# Autodesk Inventor assembly: F_Foot
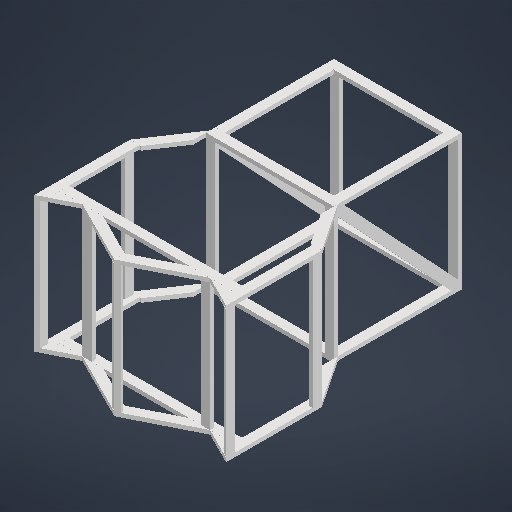
[picture p0: Inventor's stored thumbnail of the model, 512x512]
Saved by Autodesk Inventor 2027.1 (Build 311270010, 270A)
## iProperties
Created: 2025-09-08
Part Number: F_Foot
Document SubType Name: Assembly
Designer: trott
Author: trott
## Documents named in this file (11)
- C:\Users\jorda\OneDrive\Documents\GitHub\USC-ASME-TigerBurn-2026\CAD\Legs\Front Foot\F_Foot.iam
- C:\Users\jorda\OneDrive\Documents\GitHub\USC-ASME-TigerBurn-2026\CAD\Legs\Front Foot\2x4x48.ipt
- C:\Users\jorda\OneDrive\Documents\GitHub\USC-ASME-TigerBurn-2026\CAD\Legs\Front Foot\2x4x41.ipt
- C:\Users\jorda\OneDrive\Documents\GitHub\USC-ASME-TigerBurn-2026\CAD\Legs\Front Foot\2x4x65.ipt
- C:\Users\jorda\OneDrive\Documents\GitHub\USC-ASME-TigerBurn-2026\CAD\Legs\Front Foot\S_2x4x36.ipt
- C:\Users\jorda\OneDrive\Documents\GitHub\USC-ASME-TigerBurn-2026\CAD\Legs\Front Foot\S_2x4x9.503.ipt
- C:\Users\jorda\OneDrive\Documents\GitHub\USC-ASME-TigerBurn-2026\CAD\Legs\Front Foot\S_2x4x26.833.ipt
- C:\Users\jorda\OneDrive\Documents\GitHub\USC-ASME-TigerBurn-2026\CAD\Legs\Front Foot\S2_2x4x48.ipt
- C:\Users\jorda\OneDrive\Documents\GitHub\USC-ASME-TigerBurn-2026\CAD\Legs\Front Foot\S_2x4x48.ipt
- C:\Users\jorda\OneDrive\Documents\GitHub\USC-ASME-TigerBurn-2026\CAD\Legs\Front Foot\S_2x4x21.633.ipt
- C:\Users\jorda\OneDrive\Documents\GitHub\USC-ASME-TigerBurn-2026\CAD\Legs\Front Foot\S_2x4x65.795.ipt
## Components (39 placed, 10 different names)
1. 2x4x48:7 — Mate:17, Flush:23, Flush:24
2. 2x4x48:8 — Mate:18, Flush:25, Flush:26
3. S2_2x4x48:1 — Mate:19, Flush:27, Flush:28
4. S_2x4x48:1
5. S_2x4x48:2
6. 2x4x48:9 — Mate:39
7. 2x4x48:10 — Mate:36, Flush:54, Mate:42, Flush:55, Flush:56, Flush:57, Mate:43
8. S_2x4x65.795:1 — Mate:36
9. S_2x4x65.795:2 — Mate:39
10. 2x4x48:11 — Flush:54, Mate:42, Flush:55, Mate:46, Flush:62, Flush:63, Mate:47, Flush:64, Flush:65
11. 2x4x48:12 — Flush:56, Flush:57, Mate:43
12. 2x4x48:13 — Mate:44, Flush:58, Flush:59
13. 2x4x48:14 — Mate:45, Flush:60, Flush:61
14. 2x4x48:2 — Mate:44, Flush:58, Flush:59, Mate:45, Flush:60
15. 2x4x48:3
16. 2x4x48:4 — Mate:20, Flush:61
17. 2x4x48:5 — Mate:22
18. S_2x4x21.633:1
19. S_2x4x21.633:2
20. S_2x4x21.633:3
21. S_2x4x21.633:4 — Mate:20, Flush:29
22. 2x4x41:2 — Mate:47, Flush:64, Flush:65
23. 2x4x41:1 — Mate:46, Flush:62, Flush:63
24. S_2x4x36:2 — Mate:10, Flush:18, Mate:18, Flush:25, Flush:26, Flush:29, Mate:40, Flush:53
25. 2x4x65:1 — Mate:40, Flush:53, Mate:41
26. S_2x4x9.503:2 — Mate:10, Flush:18, Mate:22, Mate:41
27. S_2x4x26.833:2 — Mate:14, Flush:27
28. S_2x4x26.833:1 — Mate:13, Mate:14, Mate:19, Flush:28
29. S_2x4x9.503:1 — Mate:8, Flush:17, Mate:13
30. S_2x4x36:1 — Mate:8, Flush:17, Mate:17, Flush:23, Flush:24
31. 2x4x41:3
32. 2x4x41:4
33. S_2x4x36:3
34. 2x4x65:2
35. S_2x4x9.503:3
36. S_2x4x26.833:3
37. S_2x4x26.833:4
38. S_2x4x9.503:4
39. S_2x4x36:4
## Component patterns: (4 elements, first: 2x4x48:2), (2 elements, first: S_2x4x21.633:1 + S_2x4x21.633:2), (2 elements, first: 2x4x41:2 + 2x4x41:1 + S_2x4x36:2 + 2x4x65:1 + S_2x4x9.503:2 + S_2x4x26.833:2 + S_2x4x26.833:1 + S_2x4x9.503:1 + S_2x4x36:1)
## Relationships (41: Flush 22, Mate 19)
- Mate:8: S_2x4x9.503:1 ↔ S_2x4x36:1
- Flush:17: S_2x4x9.503:1 ↔ S_2x4x36:1
- Mate:10: S_2x4x36:2 ↔ S_2x4x9.503:2
- Flush:18: S_2x4x36:2 ↔ S_2x4x9.503:2
- Mate:13: S_2x4x26.833:1 ↔ S_2x4x9.503:1
- Mate:14: S_2x4x26.833:2 ↔ S_2x4x26.833:1
- Mate:17: 2x4x48:7 ↔ S_2x4x36:1
- Flush:23: 2x4x48:7 ↔ S_2x4x36:1
- Flush:24: 2x4x48:7 ↔ S_2x4x36:1
- Mate:18: 2x4x48:8 ↔ S_2x4x36:2
- Flush:25: 2x4x48:8 ↔ S_2x4x36:2
- Flush:26: 2x4x48:8 ↔ S_2x4x36:2
- Mate:19: S2_2x4x48:1 ↔ S_2x4x26.833:1
- Flush:27: S2_2x4x48:1 ↔ S_2x4x26.833:2
- Flush:28: S2_2x4x48:1 ↔ S_2x4x26.833:1
- Mate:20: 2x4x48:4 ↔ S_2x4x21.633:4
- Flush:29: S_2x4x21.633:4 ↔ S_2x4x36:2
- Mate:22: 2x4x48:5 ↔ S_2x4x9.503:2
- Mate:36: 2x4x48:10 ↔ S_2x4x65.795:1
- Mate:39: 2x4x48:9 ↔ S_2x4x65.795:2
- Mate:40: S_2x4x36:2 ↔ 2x4x65:1
- Flush:53: S_2x4x36:2 ↔ 2x4x65:1
- Mate:41: 2x4x65:1 ↔ S_2x4x9.503:2
- Flush:54: 2x4x48:10 ↔ 2x4x48:11
- Mate:42: 2x4x48:10 ↔ 2x4x48:11
- Flush:55: 2x4x48:10 ↔ 2x4x48:11
- Flush:56: 2x4x48:10 ↔ 2x4x48:12
- Flush:57: 2x4x48:10 ↔ 2x4x48:12
- Mate:43: 2x4x48:10 ↔ 2x4x48:12
- Mate:44: 2x4x48:13 ↔ 2x4x48:2
- Flush:58: 2x4x48:13 ↔ 2x4x48:2
- Flush:59: 2x4x48:13 ↔ 2x4x48:2
- Mate:45: 2x4x48:14 ↔ 2x4x48:2
- Flush:60: 2x4x48:14 ↔ 2x4x48:2
- Flush:61: 2x4x48:14 ↔ 2x4x48:4
- Mate:46: 2x4x48:11 ↔ 2x4x41:1
- Flush:62: 2x4x48:11 ↔ 2x4x41:1
- Flush:63: 2x4x48:11 ↔ 2x4x41:1
- Mate:47: 2x4x48:11 ↔ 2x4x41:2
- Flush:64: 2x4x48:11 ↔ 2x4x41:2
- Flush:65: 2x4x48:11 ↔ 2x4x41:2
